# Autodesk Inventor assembly: Plataforma_flotante
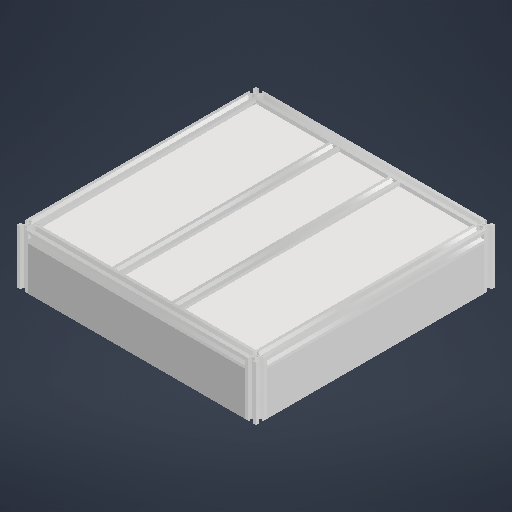
[picture p0: Inventor's stored thumbnail of the model, 512x512]
Saved by Autodesk Inventor 2026 (Build 300175050, 175E)
## iProperties
Created: 2024-02-07
Part Number: Plataforma_flotante
Document SubType Name: Assembly
Designer: diego
Mass: 53763.4 g
Surface Area: 46869.6 cm^2
Volume: 53763.4 cm^3
Author: diego
## Documents named in this file (7)
- C:\Users\habbo\OneDrive\Documents\GitHub\Tesis_Mecanismo\CAD\Plataforma_flotante\Plataforma_flotante.iam
- C:\Users\habbo\OneDrive\Documents\GitHub\Tesis_Mecanismo\CAD\Piezas Variadas\V_slots\vslot_400mm.ipt
- C:\Users\habbo\OneDrive\Documents\GitHub\Tesis_Mecanismo\CAD\Piezas Variadas\V_slots\vslot_100mm.ipt
- C:\Users\habbo\OneDrive\Documents\GitHub\Tesis_Mecanismo\CAD\Plataforma_flotante\Tapa base.ipt
- C:\Users\habbo\OneDrive\Documents\GitHub\Tesis_Mecanismo\CAD\Plataforma_flotante\Tapa lados.ipt
- C:\Users\habbo\OneDrive\Documents\GitHub\Tesis_Mecanismo\CAD\Piezas Variadas\V_slots\2020 Corner Bracket.ipt
- C:\Users\habbo\OneDrive\Documents\GitHub\Tesis_Mecanismo\CAD\Piezas Variadas\V_slots\vslot_2040_130mm.ipt
## Components (21 placed, 6 different names)
1. vslot_100mm:1 — Mate:43, Flush:62, Flush:66, Flush:67, Mate:53
2. vslot_400mm:2 — Mate:76
3. vslot_400mm:1 — Flush:61, Mate:46, Mate:54
4. vslot_100mm:3 — Flush:63, Flush:64, Mate:50
5. vslot_100mm:4 — Flush:65, Mate:52
6. vslot_400mm:4 — Mate:49
7. vslot_400mm:3 — Mate:51, Flush:68, Flush:69, Mate:75
8. vslot_100mm:5
9. Tapa lados:1 — Flush:61, Mate:43, Flush:62
10. vslot_400mm:5 — Mate:46, Mate:48, Mate:49, Mate:55, Flush:68, Mate:67, Flush:86
11. vslot_400mm:6 — Mate:48, Mate:54, Mate:55, Flush:69, Mate:68, Mate:69, Flush:87, Mate:71, Flush:92, Mate:77
12. Tapa lados:2 — Flush:65, Mate:51, Mate:52
13. Tapa lados:3 — Flush:66, Flush:67, Mate:53
14. Tapa lados:4 — Flush:63, Flush:64, Mate:50
15. 2020 Corner Bracket:1 — Mate:68, Flush:85, Flush:86, Flush:88, Flush:90
16. 2020 Corner Bracket:2 — Mate:67, Flush:85, Flush:87, Flush:89, Mate:72
17. 2020 Corner Bracket:3 — Mate:69, Flush:84, Flush:89, Mate:74, Flush:91
18. 2020 Corner Bracket:4 — Flush:84, Flush:88
19. vslot_2040_130mm:1 — Mate:71, Mate:72, Flush:90
20. vslot_2040_130mm:2 — Mate:74, Flush:91, Mate:77
21. Tapa base:1 — Flush:92, Mate:75, Mate:76
## Relationships (58: Flush 32, Mate 26)
- [Mate]: vslot_100mm:1 ↔ vslot_400mm:2
- [Mate]: vslot_100mm:1 ↔ vslot_400mm:1
- [Flush]: vslot_400mm:2 ↔ vslot_400mm:1
- [Flush]: vslot_100mm:1 ↔ vslot_400mm:1
- [Flush]: vslot_100mm:1 ↔ vslot_400mm:2
- [Flush]: vslot_100mm:1 ↔ vslot_400mm:2
- [Mate]: vslot_400mm:1 ↔ vslot_100mm:3
- [Flush]: vslot_400mm:1 ↔ vslot_100mm:3
- [Flush]: vslot_400mm:1 ↔ vslot_100mm:3
- [Mate]: vslot_100mm:4 ↔ vslot_400mm:4
- [Mate]: vslot_100mm:4 ↔ vslot_400mm:3
- [Flush]: vslot_400mm:4 ↔ vslot_400mm:3
- [Flush]: vslot_100mm:4 ↔ vslot_400mm:3
- [Flush]: vslot_100mm:4 ↔ vslot_400mm:4
- [Flush]: vslot_100mm:4 ↔ vslot_400mm:4
- [Mate]: vslot_400mm:3 ↔ vslot_100mm:5
- [Flush]: vslot_400mm:3 ↔ vslot_100mm:5
- [Flush]: vslot_400mm:3 ↔ vslot_100mm:5
- [Mate]: vslot_400mm:2 ↔ vslot_100mm:5
- [Flush]: vslot_400mm:2 ↔ vslot_100mm:4
- [Flush]: vslot_400mm:2 ↔ vslot_100mm:5
- Flush:61: vslot_400mm:1 ↔ Tapa lados:1
- Mate:43: vslot_100mm:1 ↔ Tapa lados:1
- Flush:62: vslot_100mm:1 ↔ Tapa lados:1
- Mate:46: vslot_400mm:1 ↔ vslot_400mm:5
- Mate:48 (90 mm): vslot_400mm:5 ↔ vslot_400mm:6
- Mate:49 (135 mm): vslot_400mm:4 ↔ vslot_400mm:5
- Flush:63: vslot_100mm:3 ↔ Tapa lados:4
- Flush:64: vslot_100mm:3 ↔ Tapa lados:4
- Mate:50: vslot_100mm:3 ↔ Tapa lados:4
- Flush:65: vslot_100mm:4 ↔ Tapa lados:2
- Mate:51: vslot_400mm:3 ↔ Tapa lados:2
- Mate:52: vslot_100mm:4 ↔ Tapa lados:2
- Flush:66: vslot_100mm:1 ↔ Tapa lados:3
- Flush:67: vslot_100mm:1 ↔ Tapa lados:3
- Mate:53: vslot_100mm:1 ↔ Tapa lados:3
- Mate:54: vslot_400mm:1 ↔ vslot_400mm:6
- Mate:55 (90 mm): vslot_400mm:5 ↔ vslot_400mm:6
- Flush:68: vslot_400mm:3 ↔ vslot_400mm:5
- Flush:69: vslot_400mm:3 ↔ vslot_400mm:6
- Mate:67: vslot_400mm:5 ↔ 2020 Corner Bracket:2
- Mate:68: vslot_400mm:6 ↔ 2020 Corner Bracket:1
- Mate:69: vslot_400mm:6 ↔ 2020 Corner Bracket:3
- Flush:84: 2020 Corner Bracket:3 ↔ 2020 Corner Bracket:4
- Flush:85: 2020 Corner Bracket:1 ↔ 2020 Corner Bracket:2
- Flush:86 (1.75 mm): vslot_400mm:5 ↔ 2020 Corner Bracket:1
- Flush:87 (1.75 mm): vslot_400mm:6 ↔ 2020 Corner Bracket:2
- Flush:88: 2020 Corner Bracket:1 ↔ 2020 Corner Bracket:4
- Flush:89: 2020 Corner Bracket:2 ↔ 2020 Corner Bracket:3
- Mate:71: vslot_400mm:6 ↔ vslot_2040_130mm:1
- Mate:72: 2020 Corner Bracket:2 ↔ vslot_2040_130mm:1
- Flush:90 (1.25 mm): 2020 Corner Bracket:1 ↔ vslot_2040_130mm:1
- Mate:74: 2020 Corner Bracket:3 ↔ vslot_2040_130mm:2
- Flush:91 (-1.25 mm): 2020 Corner Bracket:3 ↔ vslot_2040_130mm:2
- Flush:92 (10 mm): vslot_400mm:6 ↔ Tapa base:1
- Mate:75: vslot_400mm:3 ↔ Tapa base:1
- Mate:76: vslot_400mm:2 ↔ Tapa base:1
- Mate:77: vslot_400mm:6 ↔ vslot_2040_130mm:2
## Named parameters: d456_d444 = 0 mm, d457_d445 = 0 mm, d458_d446 = 0 mm, d459_d392 = 0 mm, d460_d393 = 0 mm, d461_d394 = 0 mm, d462_d395 = 0 mm, d478_d390 = 0 mm, d479_d391 = 0 mm
